# Autodesk Inventor assembly: assembly z
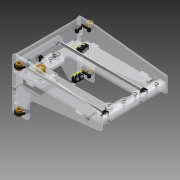
[picture p0: Inventor's stored thumbnail of the model, 180x180]
Saved by Autodesk Inventor 2015 (Build 190159000, 159)
## iProperties
Created: 2015-02-19
Part Number: assembly z
Document SubType Name: Assembly
Designer: Noa Izumi
Author: Noa Izumi
## Documents named in this file (28)
- E:\3D_Designs\Inventor\3D Printer\TinyBoy-master\src\assembly z.iam
- E:\3D_Designs\Inventor\3D Printer\TinyBoy-master\src\plastic_part_32.ipt
- E:\3D_Designs\Inventor\3D Printer\TinyBoy-master\src\plastic_part_31.ipt
- E:\3D_Designs\Inventor\3D Printer\TinyBoy-master\src\plastic_part_33.ipt
- E:\3D_Designs\Inventor\3D Printer\TinyBoy-master\src\plastic_part_34.ipt
- E:\3D_Designs\Inventor\3D Printer\TinyBoy-master\src\plastic_part_35.ipt
- E:\3D_Designs\Inventor\3D Printer\TinyBoy-master\src\plastic_part_36.ipt
- E:\3D_Designs\Inventor\3D Printer\TinyBoy-master\src\stepper_28.iam
- E:\3D_Designs\Inventor\3D Printer\TinyBoy-master\src\stepper_gear_28.ipt
- E:\3D_Designs\Inventor\3D Printer\TinyBoy-master\src\switch.ipt
- E:\3D_Designs\Inventor\3D Printer\TinyBoy-master\src\screw_M2_8.ipt
- E:\3D_Designs\Inventor\3D Printer\TinyBoy-master\src\rod_M4_130.ipt
- E:\3D_Designs\Inventor\3D Printer\TinyBoy-master\src\screw_M3_12_hex.ipt
- E:\3D_Designs\Inventor\3D Printer\TinyBoy-master\src\screw_M3_6_hex.ipt
- E:\3D_Designs\Inventor\3D Printer\TinyBoy-master\src\washer_M3.ipt
- E:\3D_Designs\Inventor\3D Printer\TinyBoy-master\src\plastic_part_37.ipt
- E:\3D_Designs\Inventor\3D Printer\TinyBoy-master\src\ring_488.ipt
- E:\3D_Designs\Inventor\3D Printer\TinyBoy-master\src\nut_M3.ipt
- E:\3D_Designs\Inventor\3D Printer\TinyBoy-master\src\screw_M3_10_hex.ipt
- E:\3D_Designs\Inventor\3D Printer\TinyBoy-master\src\plastic_part_38.ipt
- E:\3D_Designs\Inventor\3D Printer\TinyBoy-master\src\plastic_part_39.ipt
- E:\3D_Designs\Inventor\3D Printer\TinyBoy-master\src\screw_M2_5_5.ipt
- E:\3D_Designs\Inventor\3D Printer\TinyBoy-master\src\fastener_01.ipt
- E:\3D_Designs\Inventor\3D Printer\TinyBoy-master\src\fastener_02.ipt
- E:\3D_Designs\Inventor\3D Printer\TinyBoy-master\src\fastener_03.ipt
- E:\3D_Designs\Inventor\3D Printer\TinyBoy-master\src\nut_rod_M3_6.ipt
- E:\3D_Designs\Inventor\3D Printer\TinyBoy-master\src\fastener_04.ipt
- E:\3D_Designs\Inventor\3D Printer\TinyBoy-master\src\bearing_603zz.ipt
## Components (56 placed, 27 different names)
1. plastic_part_32:1 — 插入:2, 插入:3, 插入:4, 插入:5, 齊平:1, 齊平:2, 貼合:1, 齊平:3, 齊平:4, 貼合:2, 插入:8, 插入:9, 貼合:3, 齊平:6, 插入:19, 角度:1, 角度:2, 插入:39, 插入:40, 插入:43, 插入:44, 插入:45, 插入:46, 插入:47, 角度:9, 角度:10, 插入:54, 插入:55
2. plastic_part_31:1 — 齊平:1, 齊平:2, 貼合:1, 齊平:5, 插入:22, 插入:24, 角度:7, 角度:8, Mate:14, Flush:7, Mate:25, Mate:26, Mate:33, Mate:34
3. plastic_part_31:2 — 齊平:3, 齊平:4, 貼合:2, 插入:23, 插入:25, 角度:5, 角度:6, Flush:8, Mate:23, Mate:24, Mate:31, Mate:32
4. plastic_part_33:1 — 貼合:3, 齊平:5, 齊平:6, 插入:12, 插入:13, 插入:26, 插入:27, 插入:28, 插入:29, 插入:30, 插入:31, 角度:3, 角度:4, 貼合:8, 貼合:9, 貼合:10, 角度:11, 角度:12, 貼合:11, 貼合:12, 貼合:13, Angle:13
5. plastic_part_34:1 — 插入:4, 插入:5, 插入:6, 插入:7
6. plastic_part_35:1 — 插入:6, 插入:7, 插入:18, 插入:38
7. plastic_part_36:1 — 插入:14, 插入:15, 插入:18, 插入:20, 插入:21
8. stepper_28:1 [sub-assembly] — 插入:1, 插入:2, 插入:3
9. stepper_gear_28:1 — 插入:1
10. switch:1 — 插入:8, 插入:9, 插入:10, 插入:11
11. switch:2 — 插入:30, 插入:31, 插入:32, 插入:33
12. screw_M2_8:1 — 插入:10
13. screw_M2_8:2 — 插入:11
14. screw_M2_8:3 — 插入:32
15. screw_M2_8:4 — 插入:33
16. rod_M4_130:1 — 插入:12, 插入:52
17. rod_M4_130:2 — 插入:13, 插入:53
18. screw_M3_12_hex:1 — 插入:25, 插入:37
19. screw_M3_12_hex:2 — 插入:24, 插入:36
20. screw_M3_12_hex:3 — 插入:14, 插入:19
21. screw_M3_12_hex:4 — 插入:23, 插入:34
22. screw_M3_12_hex:5 — 插入:20
23. screw_M3_12_hex:6 — 插入:22, 插入:35
24. screw_M3_12_hex:7 — 插入:21
25. screw_M3_6_hex:1 — 插入:28
26. screw_M3_6_hex:2 — 插入:29
27. washer_M3:1 — 插入:17
28. washer_M3:2 — 插入:15, 插入:16
29. bearing_603zz:1 — 插入:16, 插入:17
30. plastic_part_37:1 — 插入:26, 插入:27
31. ring_488:1 — Mate:19, Mate:23, Mate:30
32. ring_488:2 — Mate:22, Mate:25, Mate:28
33. ring_488:3 — Mate:20, Mate:24, Mate:29
34. ring_488:4 — Mate:21, Mate:26, Mate:27
35. nut_M3:1 — 插入:36, 角度:4
36. nut_M3:2 — 插入:37, 角度:3
37. nut_M3:3 — 插入:35, 角度:2
38. nut_M3:4 — 插入:34, 角度:1
39. screw_M3_10_hex:1 — 插入:38
40. screw_M3_10_hex:2 — 插入:41
41. screw_M3_10_hex:3 — 插入:42
42. plastic_part_38:1 — 插入:39, 插入:40, 插入:41, 插入:42
43. plastic_part_39:1 — 插入:43, 插入:44
44. screw_M2_5_5:1 — 插入:46
45. screw_M2_5_5:2 — 插入:47
46. screw_M2_5_5:3 — 插入:45
47. fastener_01:1 — 角度:8, Mate:28, Mate:33
48. fastener_01:2 — 角度:7, Mate:27, Mate:34
49. fastener_01:3 — 角度:6, Mate:29, Mate:32
50. fastener_01:4 — 角度:5, Mate:30, Mate:31
51. fastener_02:1 — 插入:53, 角度:10
52. fastener_02:2 — 插入:52, 角度:9
53. fastener_03:1 — 貼合:8, 貼合:9, 貼合:10
54. nut_rod_M3_6:1 — 插入:54, 角度:11
55. nut_rod_M3_6:2 — 插入:55, 角度:12
56. fastener_04:1 — 貼合:11, 貼合:12, 貼合:13
## Relationships (102: Insert 51, Mate 30, Angle 13, Flush 8)
- 插入:1 [Insert]: stepper_28:1 ↔ stepper_gear_28:1
- 插入:2 [Insert]: plastic_part_32:1 ↔ stepper_28:1
- 插入:3 [Insert]: plastic_part_32:1 ↔ stepper_28:1
- 插入:4 [Insert]: plastic_part_32:1 ↔ plastic_part_34:1
- 插入:5 [Insert]: plastic_part_32:1 ↔ plastic_part_34:1
- 插入:6 [Insert]: plastic_part_34:1 ↔ plastic_part_35:1
- 插入:7 [Insert]: plastic_part_34:1 ↔ plastic_part_35:1
- 齊平:1 [Flush]: plastic_part_32:1 ↔ plastic_part_31:1
- 齊平:2 [Flush]: plastic_part_32:1 ↔ plastic_part_31:1
- 貼合:1 [Mate]: plastic_part_32:1 ↔ plastic_part_31:1
- 齊平:3 [Flush]: plastic_part_32:1 ↔ plastic_part_31:2
- 齊平:4 [Flush]: plastic_part_32:1 ↔ plastic_part_31:2
- 貼合:2 [Mate]: plastic_part_32:1 ↔ plastic_part_31:2
- 插入:8 [Insert]: plastic_part_32:1 ↔ switch:1
- 插入:9 [Insert]: plastic_part_32:1 ↔ switch:1
- 插入:10 [Insert]: switch:1 ↔ screw_M2_8:1
- 插入:11 [Insert]: switch:1 ↔ screw_M2_8:2
- 貼合:3 [Mate]: plastic_part_32:1 ↔ plastic_part_33:1
- 齊平:5 [Flush]: plastic_part_31:1 ↔ plastic_part_33:1
- 齊平:6 [Flush]: plastic_part_32:1 ↔ plastic_part_33:1
- 插入:12 [Insert] (1 mm): plastic_part_33:1 ↔ rod_M4_130:1
- 插入:13 [Insert] (1 mm): plastic_part_33:1 ↔ rod_M4_130:2
- 插入:14 [Insert]: plastic_part_36:1 ↔ screw_M3_12_hex:3
- 插入:15 [Insert]: plastic_part_36:1 ↔ washer_M3:2
- 插入:16 [Insert]: washer_M3:2 ↔ bearing_603zz:1
- 插入:17 [Insert]: washer_M3:1 ↔ bearing_603zz:1
- 插入:18 [Insert]: plastic_part_35:1 ↔ plastic_part_36:1
- 插入:19 [Insert]: plastic_part_32:1 ↔ screw_M3_12_hex:3
- 插入:20 [Insert]: plastic_part_36:1 ↔ screw_M3_12_hex:5
- 插入:21 [Insert]: plastic_part_36:1 ↔ screw_M3_12_hex:7
- 插入:22 [Insert]: plastic_part_31:1 ↔ screw_M3_12_hex:6
- 插入:23 [Insert]: plastic_part_31:2 ↔ screw_M3_12_hex:4
- 插入:24 [Insert]: plastic_part_31:1 ↔ screw_M3_12_hex:2
- 插入:25 [Insert]: plastic_part_31:2 ↔ screw_M3_12_hex:1
- 插入:26 [Insert]: plastic_part_33:1 ↔ plastic_part_37:1
- 插入:27 [Insert]: plastic_part_33:1 ↔ plastic_part_37:1
- 插入:28 [Insert]: plastic_part_33:1 ↔ screw_M3_6_hex:1
- 插入:29 [Insert]: plastic_part_33:1 ↔ screw_M3_6_hex:2
- 插入:30 [Insert]: plastic_part_33:1 ↔ switch:2
- 插入:31 [Insert]: plastic_part_33:1 ↔ switch:2
- 插入:32 [Insert]: switch:2 ↔ screw_M2_8:3
- 插入:33 [Insert]: switch:2 ↔ screw_M2_8:4
- 插入:34 [Insert]: screw_M3_12_hex:4 ↔ nut_M3:4
- 插入:35 [Insert]: screw_M3_12_hex:6 ↔ nut_M3:3
- 插入:36 [Insert]: screw_M3_12_hex:2 ↔ nut_M3:1
- 插入:37 [Insert]: screw_M3_12_hex:1 ↔ nut_M3:2
- 角度:1 [Angle] (0 deg): plastic_part_32:1 ↔ nut_M3:4
- 角度:2 [Angle] (0 deg): plastic_part_32:1 ↔ nut_M3:3
- 角度:3 [Angle] (0 deg): plastic_part_33:1 ↔ nut_M3:2
- 角度:4 [Angle] (0 deg): plastic_part_33:1 ↔ nut_M3:1
- 插入:38 [Insert]: plastic_part_35:1 ↔ screw_M3_10_hex:1
- 插入:39 [Insert]: plastic_part_32:1 ↔ plastic_part_38:1
- 插入:40 [Insert]: plastic_part_32:1 ↔ plastic_part_38:1
- 插入:41 [Insert]: screw_M3_10_hex:2 ↔ plastic_part_38:1
- 插入:42 [Insert]: screw_M3_10_hex:3 ↔ plastic_part_38:1
- 插入:43 [Insert]: plastic_part_32:1 ↔ plastic_part_39:1
- 插入:44 [Insert]: plastic_part_32:1 ↔ plastic_part_39:1
- 插入:45 [Insert]: plastic_part_32:1 ↔ screw_M2_5_5:3
- 插入:46 [Insert]: plastic_part_32:1 ↔ screw_M2_5_5:1
- 插入:47 [Insert]: plastic_part_32:1 ↔ screw_M2_5_5:2
- 角度:5 [Angle] (0 deg): plastic_part_31:2 ↔ fastener_01:4
- 角度:6 [Angle] (0 deg): plastic_part_31:2 ↔ fastener_01:3
- 角度:7 [Angle] (0 deg): plastic_part_31:1 ↔ fastener_01:2
- 角度:8 [Angle] (0 deg): plastic_part_31:1 ↔ fastener_01:1
- 插入:52 [Insert]: rod_M4_130:1 ↔ fastener_02:2
- 插入:53 [Insert]: rod_M4_130:2 ↔ fastener_02:1
- 角度:9 [Angle] (0 deg): plastic_part_32:1 ↔ fastener_02:2
- 角度:10 [Angle] (0 deg): plastic_part_32:1 ↔ fastener_02:1
- 貼合:8 [Mate]: plastic_part_33:1 ↔ fastener_03:1
- 貼合:9 [Mate]: plastic_part_33:1 ↔ fastener_03:1
- 貼合:10 [Mate]: plastic_part_33:1 ↔ fastener_03:1
- 插入:54 [Insert]: plastic_part_32:1 ↔ nut_rod_M3_6:1
- 插入:55 [Insert]: plastic_part_32:1 ↔ nut_rod_M3_6:2
- 角度:11 [Angle] (0 deg): plastic_part_33:1 ↔ nut_rod_M3_6:1
- 角度:12 [Angle] (0 deg): plastic_part_33:1 ↔ nut_rod_M3_6:2
- 貼合:11 [Mate]: plastic_part_33:1 ↔ fastener_04:1
- 貼合:12 [Mate]: plastic_part_33:1 ↔ fastener_04:1
- 貼合:13 [Mate]: plastic_part_33:1 ↔ fastener_04:1
- Mate:14: plastic_part_31:1
- Angle:13 (0 deg): plastic_part_33:1
- Flush:7 (3 mm): plastic_part_31:1
- Flush:8 (3 mm): plastic_part_31:2
- Mate:15
- Mate:16
- Mate:17
- Mate:18
- Mate:19: ring_488:1
- Mate:20: ring_488:3
- Mate:21: ring_488:4
- Mate:22: ring_488:2
- Mate:23: plastic_part_31:2 ↔ ring_488:1
- Mate:24: plastic_part_31:2 ↔ ring_488:3
- Mate:25: plastic_part_31:1 ↔ ring_488:2
- Mate:26: plastic_part_31:1 ↔ ring_488:4
- Mate:27: ring_488:4 ↔ fastener_01:2
- Mate:28: ring_488:2 ↔ fastener_01:1
- Mate:29: ring_488:3 ↔ fastener_01:3
- Mate:30: ring_488:1 ↔ fastener_01:4
- Mate:31: plastic_part_31:2 ↔ fastener_01:4
- Mate:32: plastic_part_31:2 ↔ fastener_01:3
- Mate:33: plastic_part_31:1 ↔ fastener_01:1
- Mate:34: plastic_part_31:1 ↔ fastener_01:2
